# Autodesk Inventor assembly: rs775_4_MIR
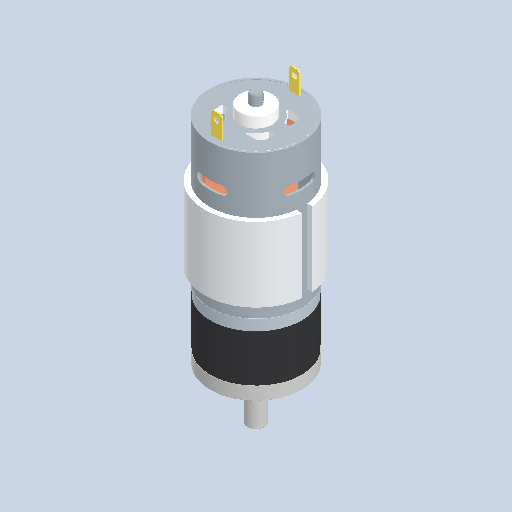
[picture p0: Inventor's stored thumbnail of the model, 512x512]
Saved by Autodesk Inventor 2025.1 (Build 291241000, 241)
## iProperties
Created: 2023-12-04
Part Number: rs775_4_MIR
Document SubType Name: Assembly
Designer: haruy
Author: fhbdh
## Documents named in this file (3)
- C:\Users\haruy\Documents\ロボコン\NHK2025\cad\nagahisa\base_weel\takagi_weel\Workspaces\作業スペース\takagi\omuni_wheel_ver3.0\parts\frequently used parts\モーター\RS775\rs775_4_MIR.iam
- C:\Users\haruy\Documents\ロボコン\NHK2025\cad\nagahisa\base_weel\takagi_weel\Workspaces\作業スペース\takagi\omuni_wheel_ver3.0\parts\frequently used parts\モーター\RS775\775_moter_MIR.ipt
- C:\Users\haruy\Documents\ロボコン\NHK2025\cad\nagahisa\base_weel\takagi_weel\Workspaces\作業スペース\takagi\omuni_wheel_ver3.0\parts\frequently used parts\モーター\RS775\IG42C-004-D8_MIR.ipt
## Components (2 placed, 2 different names)
1. 775_moter_MIR:1 — 挿入:2, 挿入:1
2. IG42C-004-D8_MIR:1 — 挿入:2, 挿入:1
## Relationships (2: Insert 2)
- 挿入:2 [Insert]: 775_moter_MIR:1 ↔ IG42C-004-D8_MIR:1
- 挿入:1 [Insert]: 775_moter_MIR:1 ↔ IG42C-004-D8_MIR:1
